# Autodesk Inventor assembly: 15inOwl
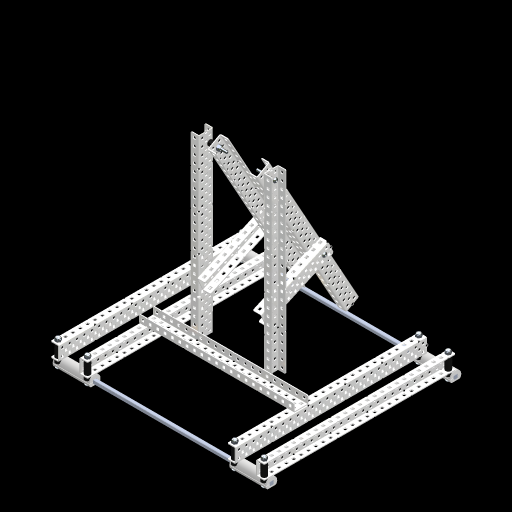
[picture p0: Inventor's stored thumbnail of the model, 512x512]
Saved by Autodesk Inventor 2024.1 (Build 281209000, 209)
## iProperties
Created: 2025-01-28
Part Number: 15inOwl
Document SubType Name: Assembly
Designer: Teddy
Author: Teddy
## Documents named in this file (20)
- C:\Users\Teddy\OneDrive\Desktop\VEX-CAD-Inventor-1.4.0\2024-25 VexGame\15inBotAub\15inOwl.iam
- C:\Users\Teddy\OneDrive\Desktop\VEX-CAD-Inventor-1.4.0\Structure\C Channel\Aluminum 1x2x1\Alu C 1x2x1x21.ipt
- C:\Users\Teddy\OneDrive\Desktop\VEX-CAD-Inventor-1.4.0\Structure\C Channel\Aluminum 1x2x1\Alu C 1x2x1x26.ipt
- C:\Users\Teddy\OneDrive\Desktop\AxleBar.ipt
- C:\Users\Teddy\OneDrive\Desktop\VEX-CAD-Inventor-1.4.0\Motion\Spacers\Spacer Nylon .375 OD\NSpacer .375 OD x .250.ipt
- C:\Users\Teddy\OneDrive\Desktop\VEX-CAD-Inventor-1.4.0\Motion\Spacers\Spacer Nylon .375 OD.ipt
- C:\Users\Teddy\OneDrive\Desktop\VEX-CAD-Inventor-1.4.0\Motion\Shaft HS\Shaft HS\Shaft HS 14.5 in.ipt
- C:\Users\Teddy\OneDrive\Desktop\VEX-CAD-Inventor-1.4.0\Motion\Shaft HS\Shaft HS.ipt
- C:\Users\Teddy\OneDrive\Desktop\VEX-CAD-Inventor-1.4.0\Structure\Hardware\Screw Steel - Star\SScrew Star Smooth 1.250.ipt
- C:\Users\Teddy\OneDrive\Desktop\VEX-CAD-Inventor-1.4.0\Structure\Hardware\Screw Steel - Star.ipt
- C:\Users\Teddy\OneDrive\Desktop\VEX-CAD-Inventor-1.4.0\Structure\Hardware\Screw Steel - Star\SScrew Star Smooth 1.750.ipt
- C:\Users\Teddy\OneDrive\Desktop\VEX-CAD-Inventor-1.4.0\Motion\Spacers\Spacer Nylon .375 OD\NSpacer .375 OD x .500.ipt
- C:\Users\Teddy\OneDrive\Desktop\VEX-CAD-Inventor-1.4.0\Motion\Spacers\Spacer Nylon .375 OD\NSpacer .375 OD x .375.ipt
- C:\Users\Teddy\OneDrive\Desktop\VEX-CAD-Inventor-1.4.0\Structure\Hardware\Nut Nylock.ipt
- C:\Users\Teddy\OneDrive\Desktop\VEX-CAD-Inventor-1.4.0\Structure\C Channel\Aluminum 1x2x1\Alu C 1x2x1x24.ipt
- C:\Users\Teddy\OneDrive\Desktop\VEX-CAD-Inventor-1.4.0\Structure\C Channel\Aluminum 1x2x1\Alu C 1x2x1x10.ipt
- C:\Users\Teddy\OneDrive\Desktop\VEX-CAD-Inventor-1.4.0\Structure\C Channel\Aluminum 1x2x1\Alu C 1x2x1x25.ipt
- C:\Users\Teddy\OneDrive\Desktop\VEX-CAD-Inventor-1.4.0\Motion\Spacers\Spacer Nylon .500 OD.ipt
- C:\Users\Teddy\OneDrive\Desktop\VEX-CAD-Inventor-1.4.0\Motion\Spacers\Spacer Nylon .500 OD\NSpacer White .500 OD x .375.ipt
- C:\Users\Teddy\OneDrive\Desktop\VEX-CAD-Inventor-1.4.0\Structure\Hardware\Screw Steel - Star\SScrew Star Smooth .750.ipt
## Components (69 placed, 15 different names)
1. Alu C 1x2x1x21:1 — Insert:1, Insert:2, Insert:3, Insert:4, Insert:57, Insert:58
2. Alu C 1x2x1x26:1 — Insert:3, Insert:4, Insert:17, Insert:20, Insert:36, Insert:44, Insert:48, Insert:49
3. Alu C 1x2x1x26:2 — Insert:1, Insert:2, Insert:13, Insert:16, Insert:41, Insert:42, Insert:53, Insert:55
4. Alu C 1x2x1x26:3 — Insert:14, Insert:15, Insert:38, Insert:40, Insert:51, Insert:56
5. Alu C 1x2x1x26:4 — Insert:18, Insert:19, Insert:26, Insert:28, Insert:45, Insert:47
6. AxleBar:1 — Insert:9, Insert:10, Insert:22, Insert:34, Insert:35
7. AxleBar:2 — Insert:11, Insert:12, Insert:21, Insert:32, Insert:33
8. AxleBar:3 — Insert:7, Insert:8, Insert:23, Insert:29, Insert:30
9. AxleBar:4 — Insert:5, Insert:6, Insert:24, Insert:25, Insert:31
10. NSpacer .375 OD x .250:1 — Insert:5, Insert:18
11. NSpacer .375 OD x .250:2 — Insert:6, Insert:17
12. NSpacer .375 OD x .250:3 — Insert:7, Insert:16
13. NSpacer .375 OD x .250:4 — Insert:8, Insert:15
14. NSpacer .375 OD x .250:5 — Insert:12, Insert:14
15. NSpacer .375 OD x .250:6 — Insert:11, Insert:13
16. NSpacer .375 OD x .250:7 — Insert:10, Insert:20
17. NSpacer .375 OD x .250:8 — Insert:9, Insert:19
18. Shaft HS 14.5 in:1 — Insert:21, Insert:22
19. Shaft HS 14.5 in:2 — Insert:23, Insert:24
20. SScrew Star Smooth 1.750:1 — Insert:25
21. NSpacer .375 OD x .500:9 — Insert:26, Insert:27
22. NSpacer .375 OD x .375:10 — Insert:27
23. NSpacer .375 OD x .375:11 — Insert:50
24. NSpacer .375 OD x .375:12 — Insert:52
25. NSpacer .375 OD x .375:13 — Insert:54
26. NSpacer .375 OD x .375:14 — Insert:39
27. NSpacer .375 OD x .375:15 — Insert:43
28. NSpacer .375 OD x .375:16 — Insert:46
29. NSpacer .375 OD x .375:17 — Insert:37
30. NSpacer .375 OD x .500:18 — Insert:49, Insert:50
31. NSpacer .375 OD x .500:19 — Insert:53, Insert:54
32. NSpacer .375 OD x .500:20 — Insert:51, Insert:52
33. NSpacer .375 OD x .500:21 — Insert:38, Insert:39
34. NSpacer .375 OD x .500:22 — Insert:36, Insert:37
35. NSpacer .375 OD x .500:23 — Insert:45, Insert:46
36. NSpacer .375 OD x .500:24 — Insert:42, Insert:43
37. SScrew Star Smooth 1.750:2 — Insert:31
38. SScrew Star Smooth 1.750:3 — Insert:30
39. SScrew Star Smooth 1.750:4 — Insert:29
40. SScrew Star Smooth 1.750:5 — Insert:33
41. SScrew Star Smooth 1.750:6 — Insert:32
42. SScrew Star Smooth 1.750:7 — Insert:34
43. SScrew Star Smooth 1.750:8 — Insert:35
44. Nut Nylock:1 — Insert:47
45. Nut Nylock:2 — Insert:44
46. Nut Nylock:3 — Insert:56
47. Nut Nylock:4 — Insert:48
48. Nut Nylock:5 — Insert:55
49. Nut Nylock:6 — Insert:41
50. Nut Nylock:7 — Insert:40
51. Nut Nylock:8 — Insert:28
52. Alu C 1x2x1x24:1 — Insert:57, Insert:59, Insert:62, Insert:72
53. Alu C 1x2x1x24:2 — Insert:58, Insert:60, Insert:61, Insert:71
54. Alu C 1x2x1x10:1 — Insert:60, Insert:65, Insert:68, Insert:70
55. Alu C 1x2x1x10:2 — Insert:59, Insert:66, Insert:67, Insert:69
56. Alu C 1x2x1x25:1 — Insert:63, Insert:65, Insert:73, Insert:76
57. Alu C 1x2x1x25:2 — Insert:64, Insert:66, Insert:74, Insert:75
58. NSpacer .375 OD x .500:25 — Insert:61, Insert:63
59. NSpacer .375 OD x .500:26 — Insert:62, Insert:64
60. NSpacer White .500 OD x .375:1 — Insert:68
61. NSpacer White .500 OD x .375:2 — Insert:67
62. SScrew Star Smooth .750:9 — Insert:70
63. SScrew Star Smooth .750:10 — Insert:69
64. SScrew Star Smooth 1.250:11 — Insert:71
65. SScrew Star Smooth 1.250:12 — Insert:72
66. Nut Nylock:9 — Insert:74
67. Nut Nylock:10 — Insert:73
68. Nut Nylock:11 — Insert:75
69. Nut Nylock:12 — Insert:76
## Relationships (76: Insert 76)
- Insert:1: Alu C 1x2x1x21:1 ↔ Alu C 1x2x1x26:2
- Insert:2: Alu C 1x2x1x21:1 ↔ Alu C 1x2x1x26:2
- Insert:3: Alu C 1x2x1x21:1 ↔ Alu C 1x2x1x26:1
- Insert:4: Alu C 1x2x1x21:1 ↔ Alu C 1x2x1x26:1
- Insert:5: AxleBar:4 ↔ NSpacer .375 OD x .250:1
- Insert:6: AxleBar:4 ↔ NSpacer .375 OD x .250:2
- Insert:7: AxleBar:3 ↔ NSpacer .375 OD x .250:3
- Insert:8: AxleBar:3 ↔ NSpacer .375 OD x .250:4
- Insert:9: AxleBar:1 ↔ NSpacer .375 OD x .250:8
- Insert:10: AxleBar:1 ↔ NSpacer .375 OD x .250:7
- Insert:11: AxleBar:2 ↔ NSpacer .375 OD x .250:6
- Insert:12: AxleBar:2 ↔ NSpacer .375 OD x .250:5
- Insert:13: Alu C 1x2x1x26:2 ↔ NSpacer .375 OD x .250:6
- Insert:14: Alu C 1x2x1x26:3 ↔ NSpacer .375 OD x .250:5
- Insert:15: Alu C 1x2x1x26:3 ↔ NSpacer .375 OD x .250:4
- Insert:16: Alu C 1x2x1x26:2 ↔ NSpacer .375 OD x .250:3
- Insert:17: Alu C 1x2x1x26:1 ↔ NSpacer .375 OD x .250:2
- Insert:18: Alu C 1x2x1x26:4 ↔ NSpacer .375 OD x .250:1
- Insert:19: Alu C 1x2x1x26:4 ↔ NSpacer .375 OD x .250:8
- Insert:20: Alu C 1x2x1x26:1 ↔ NSpacer .375 OD x .250:7
- Insert:21: AxleBar:2 ↔ Shaft HS 14.5 in:1
- Insert:22: AxleBar:1 ↔ Shaft HS 14.5 in:1
- Insert:23: AxleBar:3 ↔ Shaft HS 14.5 in:2
- Insert:24: AxleBar:4 ↔ Shaft HS 14.5 in:2
- Insert:25: AxleBar:4 ↔ SScrew Star Smooth 1.750:1
- Insert:26: Alu C 1x2x1x26:4 ↔ NSpacer .375 OD x .500:9
- Insert:27: NSpacer .375 OD x .500:9 ↔ NSpacer .375 OD x .375:10
- Insert:28: Alu C 1x2x1x26:4 ↔ Nut Nylock:8
- Insert:29: AxleBar:3 ↔ SScrew Star Smooth 1.750:4
- Insert:30: AxleBar:3 ↔ SScrew Star Smooth 1.750:3
- Insert:31: AxleBar:4 ↔ SScrew Star Smooth 1.750:2
- Insert:32: AxleBar:2 ↔ SScrew Star Smooth 1.750:6
- Insert:33: AxleBar:2 ↔ SScrew Star Smooth 1.750:5
- Insert:34: AxleBar:1 ↔ SScrew Star Smooth 1.750:7
- Insert:35: AxleBar:1 ↔ SScrew Star Smooth 1.750:8
- Insert:36: Alu C 1x2x1x26:1 ↔ NSpacer .375 OD x .500:22
- Insert:37: NSpacer .375 OD x .375:17 ↔ NSpacer .375 OD x .500:22
- Insert:38: Alu C 1x2x1x26:3 ↔ NSpacer .375 OD x .500:21
- Insert:39: NSpacer .375 OD x .375:14 ↔ NSpacer .375 OD x .500:21
- Insert:40: Alu C 1x2x1x26:3 ↔ Nut Nylock:7
- Insert:41: Alu C 1x2x1x26:2 ↔ Nut Nylock:6
- Insert:42: Alu C 1x2x1x26:2 ↔ NSpacer .375 OD x .500:24
- Insert:43: NSpacer .375 OD x .375:15 ↔ NSpacer .375 OD x .500:24
- Insert:44: Alu C 1x2x1x26:1 ↔ Nut Nylock:2
- Insert:45: Alu C 1x2x1x26:4 ↔ NSpacer .375 OD x .500:23
- Insert:46: NSpacer .375 OD x .375:16 ↔ NSpacer .375 OD x .500:23
- Insert:47: Alu C 1x2x1x26:4 ↔ Nut Nylock:1
- Insert:48: Alu C 1x2x1x26:1 ↔ Nut Nylock:4
- Insert:49: Alu C 1x2x1x26:1 ↔ NSpacer .375 OD x .500:18
- Insert:50: NSpacer .375 OD x .375:11 ↔ NSpacer .375 OD x .500:18
- Insert:51: Alu C 1x2x1x26:3 ↔ NSpacer .375 OD x .500:20
- Insert:52: NSpacer .375 OD x .375:12 ↔ NSpacer .375 OD x .500:20
- Insert:53: Alu C 1x2x1x26:2 ↔ NSpacer .375 OD x .500:19
- Insert:54: NSpacer .375 OD x .375:13 ↔ NSpacer .375 OD x .500:19
- Insert:55: Alu C 1x2x1x26:2 ↔ Nut Nylock:5
- Insert:56: Alu C 1x2x1x26:3 ↔ Nut Nylock:3
- Insert:57: Alu C 1x2x1x21:1 ↔ Alu C 1x2x1x24:1
- Insert:58: Alu C 1x2x1x21:1 ↔ Alu C 1x2x1x24:2
- Insert:59: Alu C 1x2x1x24:1 ↔ Alu C 1x2x1x10:2
- Insert:60: Alu C 1x2x1x24:2 ↔ Alu C 1x2x1x10:1
- Insert:61: Alu C 1x2x1x24:2 ↔ NSpacer .375 OD x .500:25
- Insert:62: Alu C 1x2x1x24:1 ↔ NSpacer .375 OD x .500:26
- Insert:63: Alu C 1x2x1x25:1 ↔ NSpacer .375 OD x .500:25
- Insert:64: Alu C 1x2x1x25:2 ↔ NSpacer .375 OD x .500:26
- Insert:65: Alu C 1x2x1x10:1 ↔ Alu C 1x2x1x25:1
- Insert:66: Alu C 1x2x1x10:2 ↔ Alu C 1x2x1x25:2
- Insert:67: Alu C 1x2x1x10:2 ↔ NSpacer White .500 OD x .375:2
- Insert:68: Alu C 1x2x1x10:1 ↔ NSpacer White .500 OD x .375:1
- Insert:69: Alu C 1x2x1x10:2 ↔ SScrew Star Smooth .750:10
- Insert:70: Alu C 1x2x1x10:1 ↔ SScrew Star Smooth .750:9
- Insert:71: Alu C 1x2x1x24:2 ↔ SScrew Star Smooth 1.250:11
- Insert:72: Alu C 1x2x1x24:1 ↔ SScrew Star Smooth 1.250:12
- Insert:73: Alu C 1x2x1x25:1 ↔ Nut Nylock:10
- Insert:74: Alu C 1x2x1x25:2 ↔ Nut Nylock:9
- Insert:75: Alu C 1x2x1x25:2 ↔ Nut Nylock:11
- Insert:76: Alu C 1x2x1x25:1 ↔ Nut Nylock:12
